# Autodesk Inventor assembly: Vertical Strut
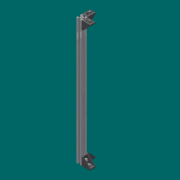
[picture p0: Inventor's stored thumbnail of the model, 180x180]
Saved by Autodesk Inventor 2016 (Build 200138000, 138)
## iProperties
Created: 2015-06-02
Part Number: Vertical Strut
Document SubType Name: Assembly
Designer: Sawaiz Syed
Author: Sawaiz Syed
## Documents named in this file (4)
- C:\Users\Sawaiz\Documents\data\projects\cncBlackBox\frame\Vertical Strut.iam
- C:\Users\Sawaiz\Documents\data\projects\cncBlackBox\frame\HFS5-2020-460.ipt
- C:\Users\Admin\SkyDrive\Classes\Reaserch\Black Box\HFS5-2020.ipt
- C:\Users\Sawaiz\Documents\data\projects\cncBlackBox\frame\angleBracket.iam
## Components (5 placed, 2 different names)
1. HFS5-2020-460:1 — Mate:1, Mate:2, Flush:3, Flush:4, Flush:6, Flush:8, Flush:9, Flush:10
2. angleBracket:1 [sub-assembly] — Flush:2, Flush:7, Flush:9
3. angleBracket:2 [sub-assembly] — Flush:1, Flush:7, Flush:8, Flush:10
4. angleBracket:3 [sub-assembly] — Flush:2, Mate:1, Flush:4, Flush:5
5. angleBracket:4 [sub-assembly] — Flush:1, Mate:2, Flush:3, Flush:5, Flush:6
## Relationships (12: Flush 10, Mate 2)
- Flush:1: angleBracket:2 ↔ angleBracket:4
- Flush:2: angleBracket:1 ↔ angleBracket:3
- Mate:1: HFS5-2020-460:1 ↔ angleBracket:3
- Mate:2: HFS5-2020-460:1 ↔ angleBracket:4
- Flush:3: HFS5-2020-460:1 ↔ angleBracket:4
- Flush:4: HFS5-2020-460:1 ↔ angleBracket:3
- Flush:5: angleBracket:3 ↔ angleBracket:4
- Flush:6: HFS5-2020-460:1 ↔ angleBracket:4
- Flush:7: angleBracket:1 ↔ angleBracket:2
- Flush:8: HFS5-2020-460:1 ↔ angleBracket:2
- Flush:9: HFS5-2020-460:1 ↔ angleBracket:1
- Flush:10: HFS5-2020-460:1 ↔ angleBracket:2
